# Autodesk Inventor assembly: Z axis motor mount sub-assembly
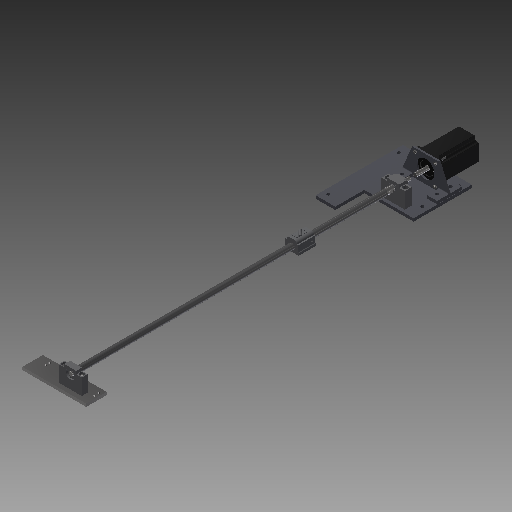
[picture p0: Inventor's stored thumbnail of the model, 512x512]
Saved by Autodesk Inventor 2018 (Build 220112000, 112)
## iProperties
Created: 2018-03-20
Part Number: Z axis motor mount sub-assembly
Document SubType Name: Assembly
Designer: M224826
Author: M224826
## Documents named in this file (8)
- C:\Users\P300023\Documents\GitHub\CNC-Lathe-CAD2.0\CNC Lathe Project\Project Files\Updated Z axis\Z axis motor mount sub-assembly.iam
- C:\Users\P300023\Documents\GitHub\CNC-Lathe-CAD2.0\CNC Lathe Project\Project Files\Updated Z axis\Motor Support Fin.ipt
- C:\Users\P300023\Documents\GitHub\CNC-Lathe-CAD2.0\CNC Lathe Project\Project Files\Updated Z axis\SUPPORT MAIN FRAME MOTOR-BALL SCREW-REV-B.ipt
- C:\Users\P300023\Documents\GitHub\CNC-Lathe-CAD2.0\CNC Lathe Project\Project Files\Servo Motor\Servo Motor.iam
- C:\Users\P300023\Documents\GitHub\CNC-Lathe-CAD2.0\CNC Lathe Project\Project Files\Updated Z axis\AIS2016\Z-AxisLong-Shaft-Final.iam
- C:\Users\P300023\Documents\GitHub\CNC-Lathe-CAD2.0\CNC Lathe Project\Project Files\Updated Z axis\Ball screw right hand support.ipt
- C:\Users\P300023\Documents\Inventor\Content Center Files\R2018\en-US\U 2494(2)\Unbrako - M10 x  45(7).ipt
- C:\Users\P300023\Documents\Inventor\Content Center Files\R2018\en-US\U 2494(2)\Unbrako - M6 x  35(7).ipt
## Components (13 placed, 7 different names)
1. Motor Support Fin:1 — Mate:3, Mate:5, Angle:1, Mate:6, Mate:7, Mate:8, Insert:1, Insert:2, Insert:3, Insert:4
2. SUPPORT MAIN FRAME MOTOR-BALL SCREW-REV-B:1 — Flush:1, Flush:2, Flush:3, Mate:3, Mate:6, Mate:7, Mate:9, Mate:10, Mate:11
3. Servo Motor:1 [sub-assembly] — Mate:5, Angle:1, Mate:8
4. Z-AxisLong-Shaft-Final:1 [sub-assembly] — Mate:9, Mate:10, Mate:11, Mate:14, Mate:15, Mate:16, Mate:18, Mate:20, Mate:21, Mate:22, Mate:23, Mate:24
5. Ball screw right hand support:1 — Mate:14, Mate:15, Mate:16, Mate:17, Mate:19
6. Unbrako Hex Socket Cap (Flat Head Height) - Metric M10 x 45:1 — Mate:17, Mate:18
7. Unbrako Hex Socket Cap (Flat Head Height) - Metric M10 x 45:2 — Mate:19, Mate:20
8. Unbrako Hex Socket Cap (Flat Head Height) - Metric M10 x 45:3 — Mate:21, Mate:22
9. Unbrako Hex Socket Cap (Flat Head Height) - Metric M10 x 45:4 — Mate:23, Mate:24
10. Unbrako Hex Socket Cap (Flat Head Height) - Metric M6 x 35:1 — Insert:1
11. Unbrako Hex Socket Cap (Flat Head Height) - Metric M6 x 35:2 — Insert:2
12. Unbrako Hex Socket Cap (Flat Head Height) - Metric M6 x 35:3 — Insert:3
13. Unbrako Hex Socket Cap (Flat Head Height) - Metric M6 x 35:4 — Insert:4
## Relationships (27: Mate 19, Insert 4, Flush 3, Angle 1)
- Flush:1: SUPPORT MAIN FRAME MOTOR-BALL SCREW-REV-B:1
- Flush:2: SUPPORT MAIN FRAME MOTOR-BALL SCREW-REV-B:1
- Flush:3: SUPPORT MAIN FRAME MOTOR-BALL SCREW-REV-B:1
- Mate:3: Motor Support Fin:1 ↔ SUPPORT MAIN FRAME MOTOR-BALL SCREW-REV-B:1
- Mate:5: Motor Support Fin:1 ↔ Servo Motor:1
- Angle:1 (90 deg): Motor Support Fin:1 ↔ Servo Motor:1
- Mate:6: Motor Support Fin:1 ↔ SUPPORT MAIN FRAME MOTOR-BALL SCREW-REV-B:1
- Mate:7: Motor Support Fin:1 ↔ SUPPORT MAIN FRAME MOTOR-BALL SCREW-REV-B:1
- Mate:8: Motor Support Fin:1 ↔ Servo Motor:1
- Mate:9: SUPPORT MAIN FRAME MOTOR-BALL SCREW-REV-B:1 ↔ Z-AxisLong-Shaft-Final:1
- Mate:10: SUPPORT MAIN FRAME MOTOR-BALL SCREW-REV-B:1 ↔ Z-AxisLong-Shaft-Final:1
- Mate:11: SUPPORT MAIN FRAME MOTOR-BALL SCREW-REV-B:1 ↔ Z-AxisLong-Shaft-Final:1
- Mate:14: Z-AxisLong-Shaft-Final:1 ↔ Ball screw right hand support:1
- Mate:15: Z-AxisLong-Shaft-Final:1 ↔ Ball screw right hand support:1
- Mate:16: Z-AxisLong-Shaft-Final:1 ↔ Ball screw right hand support:1
- Mate:17: Ball screw right hand support:1 ↔ Unbrako Hex Socket Cap (Flat Head Height) - Metric M10 x 45:1
- Mate:18: Z-AxisLong-Shaft-Final:1 ↔ Unbrako Hex Socket Cap (Flat Head Height) - Metric M10 x 45:1
- Mate:19: Ball screw right hand support:1 ↔ Unbrako Hex Socket Cap (Flat Head Height) - Metric M10 x 45:2
- Mate:20: Z-AxisLong-Shaft-Final:1 ↔ Unbrako Hex Socket Cap (Flat Head Height) - Metric M10 x 45:2
- Mate:21: Z-AxisLong-Shaft-Final:1 ↔ Unbrako Hex Socket Cap (Flat Head Height) - Metric M10 x 45:3
- Mate:22: Z-AxisLong-Shaft-Final:1 ↔ Unbrako Hex Socket Cap (Flat Head Height) - Metric M10 x 45:3
- Mate:23: Z-AxisLong-Shaft-Final:1 ↔ Unbrako Hex Socket Cap (Flat Head Height) - Metric M10 x 45:4
- Mate:24: Z-AxisLong-Shaft-Final:1 ↔ Unbrako Hex Socket Cap (Flat Head Height) - Metric M10 x 45:4
- Insert:1: Motor Support Fin:1 ↔ Unbrako Hex Socket Cap (Flat Head Height) - Metric M6 x 35:1
- Insert:2: Motor Support Fin:1 ↔ Unbrako Hex Socket Cap (Flat Head Height) - Metric M6 x 35:2
- Insert:3: Motor Support Fin:1 ↔ Unbrako Hex Socket Cap (Flat Head Height) - Metric M6 x 35:3
- Insert:4: Motor Support Fin:1 ↔ Unbrako Hex Socket Cap (Flat Head Height) - Metric M6 x 35:4
